# Autodesk Inventor assembly: 1FullPin
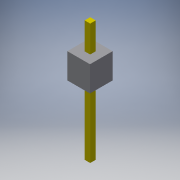
[picture p0: Inventor's stored thumbnail of the model, 180x180]
Saved by Autodesk Inventor 2019 (Build 230136000, 136)
## iProperties
Created: 2019-07-16
Part Number: 1FullPin
Document SubType Name: Assembly
Designer: james
Author: james
## Documents named in this file (3)
- F:\JimsDesign\P1001-16bit-CPU\P1001-001 - 16bit CPU\P1001-001-210 - CAD Library\1FullPin.iam
- F:\JimsDesign\P1001-16bit-CPU\P1001-001 - 16bit CPU\P1001-001-210 - CAD Library\HeaderBlock.ipt
- F:\JimsDesign\P1001-16bit-CPU\P1001-001 - 16bit CPU\P1001-001-210 - CAD Library\HeaderPin.ipt
## Components (2 placed, 2 different names)
1. HeaderBlock:1 — Mate:1, Mate:2, Flush:1
2. HeaderPin:1 — Mate:1, Mate:2, Flush:1
## Relationships (3: Mate 2, Flush 1)
- Mate:1: HeaderBlock:1 ↔ HeaderPin:1
- Mate:2: HeaderBlock:1 ↔ HeaderPin:1
- Flush:1 (3 mm): HeaderBlock:1 ↔ HeaderPin:1
